# Autodesk Inventor assembly: cellSTORM_v5_microsocpe
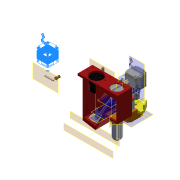
[picture p0: Inventor's stored thumbnail of the model, 180x180]
Saved by Autodesk Inventor 2022 (Build 260153000, 153)
## iProperties
Created: 2020-04-25
Part Number: cellSTORM_v5_microsocpe
Document SubType Name: Assembly
Designer: diederichbenedict
Author: diederichbenedict
## Documents named in this file (15)
- C:\Users\Muriel\Documents\GitHub\cellstorm\INVENTOR\cellSTORM_v5_microsocpe.iam
- C:\Users\Muriel\Documents\GitHub\cellstorm\INVENTOR\00_Eyepiece_20x_WF.ipt
- C:\Users\Muriel\Documents\GitHub\cellstorm\INVENTOR\cellSTORM_lightpath.ipt
- C:\Users\Muriel\Documents\GitHub\cellstorm\INVENTOR\PF10-03-P01-Step.ipt
- C:\Users\Muriel\Documents\GitHub\cellstorm\INVENTOR\cellSTORM_v5_opticalstage.ipt
- C:\Users\Muriel\Documents\GitHub\cellstorm\INVENTOR\00_Motorcoupling_5mm_M3.ipt
- C:\Users\Muriel\Documents\GitHub\cellstorm\INVENTOR\30_Cube_Z_Focus_MGN12_NEMA_slide_part2.ipt
- C:\Users\Muriel\Documents\GitHub\cellstorm\INVENTOR\00_NEMA11.ipt
- C:\Users\Muriel\Documents\GitHub\cellstorm\INVENTOR\00_bearing_ball_2mm.ipt
- C:\Users\Muriel\Documents\GitHub\cellstorm\INVENTOR\30_Cube_Z_Focus_Drylin_NEMA_slide_part1.ipt
- C:\Users\Muriel\Documents\GitHub\cellstorm\INVENTOR\30_Cube_Z_Focus_MGN_NEMA_rail.ipt
- C:\Users\Muriel\Documents\GitHub\cellstorm\INVENTOR\00_MGN12H, LINEAR GUIDE BLOCK.ipt
- C:\Users\Muriel\Documents\GitHub\cellstorm\INVENTOR\00_Microscope_Objective.ipt
- C:\Users\Muriel\Documents\GitHub\cellstorm\INVENTOR\00_F6SS088-Step.ipt
- C:\Users\Muriel\Documents\GitHub\cellstorm\INVENTOR\00_F6SSN2P-Step.ipt
## Components (16 placed, 14 different names)
1. 00_Motorcoupling_5mm_M3:1 — Einfügen:6
2. 00_bearing_ball_2mm:1
3. 30_Cube_Z_Focus_Drylin_NEMA_slide_part1:1 — Passend:14, Passend:15, Passend:17
4. 00_bearing_ball_2mm:2
5. 30_Cube_Z_Focus_MGN_NEMA_rail:1 — Passend:7, Passend:8
6. 00_MGN12H, LINEAR GUIDE BLOCK:1 — Passend:7, Passend:8, Passend:12, Fluchtend:7
7. 00_Microscope_Objective:1 — Einfügen:5, Einfügen:10, Passend:19
8. 30_Cube_Z_Focus_MGN12_NEMA_slide_part2:1 — Passend:12, Fluchtend:7, Einfügen:5, Passend:14, Passend:15, Passend:16, Winkel:1, Passend:17, Einfügen:10
9. 00_NEMA11:1 — Passend:16, Winkel:1, Einfügen:6, Angle:2
10. 00_F6SS088-Step:1
11. 00_F6SSN2P-Step:1
12. cellSTORM_v5_opticalstage:1 — Angle:2, Einfügen:11
13. PF10-03-P01-Step:3 — Passend:20
14. PF10-03-P01-Step:4
15. 00_Eyepiece_20x_WF:1 — Einfügen:11, Passend:18
16. cellSTORM_lightpath:2 — Passend:18, Passend:19, Passend:20
## Relationships (17: Mate 10, Insert 4, Angle 2, Flush 1)
- Passend:7 [Mate]: 30_Cube_Z_Focus_MGN_NEMA_rail:1 ↔ 00_MGN12H, LINEAR GUIDE BLOCK:1
- Passend:8 [Mate] (0.1 mm): 30_Cube_Z_Focus_MGN_NEMA_rail:1 ↔ 00_MGN12H, LINEAR GUIDE BLOCK:1
- Passend:12 [Mate]: 00_MGN12H, LINEAR GUIDE BLOCK:1 ↔ 30_Cube_Z_Focus_MGN12_NEMA_slide_part2:1
- Fluchtend:7 [Flush]: 00_MGN12H, LINEAR GUIDE BLOCK:1 ↔ 30_Cube_Z_Focus_MGN12_NEMA_slide_part2:1
- Einfügen:5 [Insert]: 00_Microscope_Objective:1 ↔ 30_Cube_Z_Focus_MGN12_NEMA_slide_part2:1
- Passend:14 [Mate]: 30_Cube_Z_Focus_Drylin_NEMA_slide_part1:1 ↔ 30_Cube_Z_Focus_MGN12_NEMA_slide_part2:1
- Passend:15 [Mate]: 30_Cube_Z_Focus_Drylin_NEMA_slide_part1:1 ↔ 30_Cube_Z_Focus_MGN12_NEMA_slide_part2:1
- Passend:16 [Mate]: 30_Cube_Z_Focus_MGN12_NEMA_slide_part2:1 ↔ 00_NEMA11:1
- Winkel:1 [Angle] (180 deg): 30_Cube_Z_Focus_MGN12_NEMA_slide_part2:1 ↔ 00_NEMA11:1
- Passend:17 [Mate] (1 mm): 30_Cube_Z_Focus_Drylin_NEMA_slide_part1:1 ↔ 30_Cube_Z_Focus_MGN12_NEMA_slide_part2:1
- Einfügen:6 [Insert] (-5 mm): 00_Motorcoupling_5mm_M3:1 ↔ 00_NEMA11:1
- Angle:2 (0 deg): 00_NEMA11:1 ↔ cellSTORM_v5_opticalstage:1
- Einfügen:10 [Insert]: 00_Microscope_Objective:1 ↔ 30_Cube_Z_Focus_MGN12_NEMA_slide_part2:1
- Einfügen:11 [Insert]: cellSTORM_v5_opticalstage:1 ↔ 00_Eyepiece_20x_WF:1
- Passend:18 [Mate]: 00_Eyepiece_20x_WF:1 ↔ cellSTORM_lightpath:2
- Passend:19 [Mate]: 00_Microscope_Objective:1 ↔ cellSTORM_lightpath:2
- Passend:20 [Mate]: PF10-03-P01-Step:3 ↔ cellSTORM_lightpath:2
